# Autodesk Inventor assembly: Vertical wing
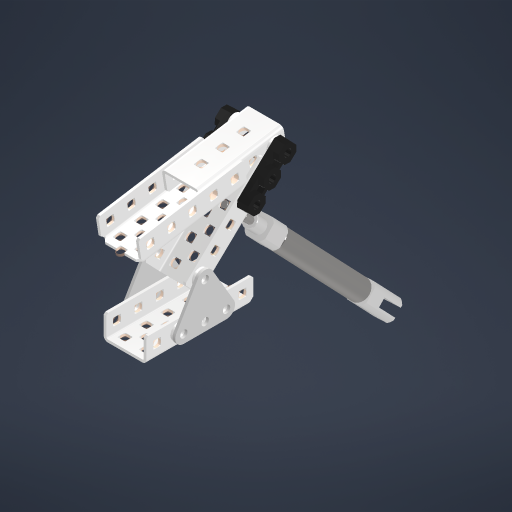
[picture p0: Inventor's stored thumbnail of the model, 512x512]
Saved by Autodesk Inventor 2023.4 (Build 274418000, 418)
## iProperties
Created: 2024-01-30
Part Number: Vertical wing
Document SubType Name: Assembly
Designer: diego
Author: diego
## Documents named in this file (8)
- C:\Users\diego\OneDrive\Documents\GitHub\2024-599Z\2024-599Z\Cad\NEW Wings\Vertical wing.iam
- C:\Users\diego\OneDrive\Documents\GitHub\2024-599Z\2024-599Z\Cad\Library\VEX-CAD-Inventor-1.4.0\Structure\Gussets\C Channel Coupler.ipt
- C:\Users\diego\OneDrive\Documents\GitHub\2024-599Z\2024-599Z\Cad\Library\VEX-CAD-Inventor-1.4.0\Structure\C Channel\Aluminum 1x2x1\Alu C 1x2x1x5.ipt
- C:\Users\diego\OneDrive\Documents\GitHub\2024-599Z\2024-599Z\Cad\NEW CNC Poly\Wing poly connection.ipt
- C:\Users\diego\OneDrive\Documents\GitHub\2024-599Z\2024-599Z\Cad\Library\VEX-CAD-Inventor-1.4.0\Motion\Spacers\Washer Teflon\TWasher .375 OD x .06250.ipt
- C:\Users\diego\OneDrive\Documents\GitHub\2024-599Z\2024-599Z\Cad\Library\VEX-CAD-Inventor-1.4.0\Motion\Spacers\Washer Teflon.ipt
- C:\Users\diego\OneDrive\Documents\GitHub\2024-599Z\2024-599Z\Cad\Library\VEX-CAD-Inventor-1.4.0\Motion\Shaft LS\Bearing Flat.ipt
- C:\Users\diego\OneDrive\Documents\GitHub\2024-599Z\2024-599Z\Cad\Library\VEX-CAD-Inventor-1.4.0\Motion\Pneumatics\Double Acting Piston.iam
## Components (17 placed, 6 different names)
1. C Channel Coupler:1 — Insert:23, Insert:24, Insert:25, Insert:26
2. Alu C 1x2x1x5:1 — Insert:11, Insert:12, Insert:13, Insert:14
3. Wing poly connection:1 — Insert:5, Insert:7, Insert:8
4. Wing poly connection:2 — Insert:6, Insert:9, Insert:10
5. Alu C 1x2x1x5:2 — Insert:15, Insert:16, Insert:17, Insert:18, Insert:19, Insert:20, Insert:27
6. TWasher .375 OD x .06250:1 — Insert:6, Insert:15
7. TWasher .375 OD x .06250:2 — Insert:5, Insert:16
8. TWasher .375 OD x .06250:3 — Insert:7, Insert:14
9. TWasher .375 OD x .06250:4 — Insert:8, Insert:13
10. TWasher .375 OD x .06250:5 — Insert:9, Insert:11
11. TWasher .375 OD x .06250:6 — Insert:10, Insert:12
12. Bearing Flat:1 — Insert:17, Insert:18, Insert:21
13. Bearing Flat:2 — Insert:19, Insert:20, Insert:22
14. TWasher .375 OD x .06250:7 — Insert:21, Insert:23
15. TWasher .375 OD x .06250:8 — Insert:22, Insert:24
16. Alu C 1x2x1x5:3 — Insert:25, Insert:26
17. Double Acting Piston:1 [sub-assembly] — Insert:27
## Relationships (23: Insert 23)
- Insert:5: Wing poly connection:1 ↔ TWasher .375 OD x .06250:2
- Insert:6: Wing poly connection:2 ↔ TWasher .375 OD x .06250:1
- Insert:7: Wing poly connection:1 ↔ TWasher .375 OD x .06250:3
- Insert:8: Wing poly connection:1 ↔ TWasher .375 OD x .06250:4
- Insert:9: Wing poly connection:2 ↔ TWasher .375 OD x .06250:5
- Insert:10: Wing poly connection:2 ↔ TWasher .375 OD x .06250:6
- Insert:11: Alu C 1x2x1x5:1 ↔ TWasher .375 OD x .06250:5
- Insert:12: Alu C 1x2x1x5:1 ↔ TWasher .375 OD x .06250:6
- Insert:13: Alu C 1x2x1x5:1 ↔ TWasher .375 OD x .06250:4
- Insert:14: Alu C 1x2x1x5:1 ↔ TWasher .375 OD x .06250:3
- Insert:15: Alu C 1x2x1x5:2 ↔ TWasher .375 OD x .06250:1
- Insert:16: Alu C 1x2x1x5:2 ↔ TWasher .375 OD x .06250:2
- Insert:17: Alu C 1x2x1x5:2 ↔ Bearing Flat:1
- Insert:18: Alu C 1x2x1x5:2 ↔ Bearing Flat:1
- Insert:19: Alu C 1x2x1x5:2 ↔ Bearing Flat:2
- Insert:20: Alu C 1x2x1x5:2 ↔ Bearing Flat:2
- Insert:21: Bearing Flat:1 ↔ TWasher .375 OD x .06250:7
- Insert:22: Bearing Flat:2 ↔ TWasher .375 OD x .06250:8
- Insert:23: C Channel Coupler:1 ↔ TWasher .375 OD x .06250:7
- Insert:24: C Channel Coupler:1 ↔ TWasher .375 OD x .06250:8
- Insert:25: C Channel Coupler:1 ↔ Alu C 1x2x1x5:3
- Insert:26: C Channel Coupler:1 ↔ Alu C 1x2x1x5:3
- Insert:27: Alu C 1x2x1x5:2 ↔ Double Acting Piston:1
